# Autodesk Inventor assembly: P1704_E001
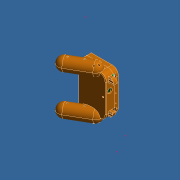
[picture p0: Inventor's stored thumbnail of the model, 180x180]
Saved by Autodesk Inventor 2019 (Build 230136000, 136)
## iProperties
Created: 2019-04-29
Part Number: P1704_E001
Material: Générique
Document SubType Name: Assembly
Designer: Joan.MAILLARD
Author: Joan.MAILLARD
## Documents named in this file (19)
- P:\projet_manette\manette\06_Dessins\2019\Manette universelle\P1704_E001.iam
- P:\projet_manette\manette\06_Dessins\2019\Manette universelle\P1704_001_basManette.ipt
- P:\projet_manette\manette\06_Dessins\2019\Manette universelle\P1704_006_gachette.ipt
- P:\projet_manette\manette\06_Dessins\2019\Manette universelle\P1704_007_guideRessort.ipt
- P:\projet_manette\manette\06_Dessins\2019\Manette universelle\P1704_002_mainDroiteInterieur.ipt
- P:\projet_manette\manette\06_Dessins\2019\Manette universelle\P1704_003_mainGaucheInterieur.ipt
- P:\projet_manette\manette\06_Dessins\2019\Manette universelle\P1704_009_slider.ipt
- P:\projet_manette\manette\06_Dessins\2019\Manette universelle\P1704_011_4buttonPCB.ipt
- P:\projet_manette\manette\06_Dessins\2019\Manette universelle\P1704_010_startSelectPCB.ipt
- P:\projet_manette\manette\06_Dessins\2019\Manette universelle\P1704_012_joystick.ipt
- P:\projet_manette\manette\06_Dessins\2019\Manette universelle\P1704_014_Display.ipt
- P:\projet_manette\manette\06_Dessins\2019\Manette universelle\P1704_015_rumble.ipt
- P:\projet_manette\manette\06_Dessins\2019\Manette universelle\P1704_008_pcb.ipt
- P:\projet_manette\manette\06_Dessins\2019\Manette universelle\P1704_018_hautManette.ipt
- P:\projet_manette\manette\06_Dessins\2019\Manette universelle\P1704_E003_button.iam
- P:\projet_manette\manette\06_Dessins\2019\Manette universelle\P1704_016_Button.ipt
- P:\projet_manette\manette\06_Dessins\2019\Manette universelle\P1704_019_button_triangle_cap.ipt
- P:\projet_manette\manette\06_Dessins\2019\Manette universelle\P1704_013_Switch.ipt
- P:\projet_manette\manette\06_Dessins\2019\Manette universelle\P1704_004_mainDroiteExterieur.ipt
## Components (37 placed, 18 different names)
1. P1704_001_basManette:1 — Placage:20, Placage:22, Placage:24, Placage:26, Placage:27, Placage:30, Placage:31, Placage:32, Placage:33, Placage:34, Placage:35, Placage:38, Placage:41, Placage:42, Placage:43, Placage:49, Affleurement:4, Affleurement:5, Placage:97, Affleurement:6, Placage:98, Placage:99, Placage:100, Placage:101, Placage:102, Placage:103, Placage:104, Placage:110, Placage:113, Placage:115, Placage:116, Placage:117, Placage:120
2. P1704_006_gachette:1 — Rotation:2, Glissière:4, Placage:26, Placage:27, Affleurement:1
3. P1704_006_gachette:2 — Rotation:1, Glissière:3, Affleurement:7, Placage:120
4. P1704_007_guideRessort:1 — Rotation:1
5. P1704_007_guideRessort:2 — Rotation:2
6. P1704_002_mainDroiteInterieur:1 — Placage:110, Placage:114, Placage:118
7. P1704_003_mainGaucheInterieur:1 — Placage:104, Placage:111, Placage:112
8. P1704_009_slider:1 — Glissière:3, Affleurement:7
9. P1704_009_slider:2 — Glissière:4, Affleurement:1
10. manette_2019_boutons.kicad_pcb_Contour:1 — Placage:22, Placage:52, Placage:53, Placage:54, Placage:56, Angle:1, Angle:2, Placage:57, Placage:58, Placage:59, Placage:60, Angle:3, Placage:61, Placage:62, Placage:63, Angle:4, Placage:64, Placage:65, Affleurement:6
11. manette_2019_boutons.kicad_pcb_Contour:2 — Placage:20, Placage:66, Placage:67, Placage:68, Placage:69, Placage:70, Angle:5, Angle:6, Angle:7, Angle:8, Placage:71, Placage:72, Placage:73, Placage:74, Placage:75, Placage:76, Placage:77, Angle:9, Angle:10, Angle:11, Angle:12, Placage:86, Placage:97
12. Manette_2019_PCB_Central.kicad_pcb_Contour:1 — Placage:24, Placage:87, Placage:88, Placage:89, Placage:90, Placage:91, Angle:13, Angle:14, Placage:92, Placage:93, Angle:15, Placage:98
13. P1704_012_joystick:1 — Placage:30, Placage:31, Placage:48
14. P1704_012_joystick:2 — Placage:32, Placage:33, Placage:47
15. P1704_014_Display:1 — Placage:38, Placage:50, Placage:96
16. P1704_015_rumble:1 — Placage:34, Placage:102
17. P1704_015_rumble:2 — Placage:35, Placage:103
18. manette_2019.kicad_pcb_Contour:1 — Placage:41, Placage:42, Placage:43, Placage:47, Placage:48
19. P1704_018_hautManette:1 — Placage:49, Affleurement:4, Affleurement:5, Placage:50, Placage:65, Placage:86, Placage:87, Placage:96
20. P1704_E003_button:1 [sub-assembly] — Placage:56, Angle:2, Placage:57, Placage:58
21. P1704_E003_button:2 [sub-assembly] — Placage:52, Placage:53, Placage:54, Angle:1
22. P1704_E003_button:3 [sub-assembly] — Placage:59, Placage:63, Angle:4, Placage:64
23. P1704_E003_button:4 [sub-assembly] — Placage:60, Angle:3, Placage:61, Placage:62
24. P1704_016_Button:1 — Placage:68, Angle:7, Placage:76, Placage:77, Placage:84, Placage:85
25. P1704_016_Button:2 — Placage:66, Angle:8, Placage:74, Placage:75, Placage:82, Placage:83
26. P1704_016_Button:3 — Placage:69, Angle:6, Placage:72, Placage:73, Placage:80, Placage:81
27. P1704_016_Button:4 — Placage:67, Placage:70, Angle:5, Placage:71, Placage:78, Placage:79
28. P1704_019_button_triangle_cap:1 — Placage:82, Placage:83, Angle:12
29. P1704_019_button_triangle_cap:2 — Placage:84, Placage:85, Angle:11
30. P1704_019_button_triangle_cap:3 — Placage:78, Placage:79, Angle:10
31. P1704_019_button_triangle_cap:4 — Placage:80, Placage:81, Angle:9
32. P1704_019_button_triangle_cap:5 — Placage:94, Placage:95, Angle:15
33. P1704_E003_button:5 [sub-assembly] — Placage:89, Placage:91, Angle:13, Placage:92
34. P1704_016_Button:5 — Placage:88, Placage:90, Angle:14, Placage:93, Placage:94, Placage:95
35. P1704_013_Switch:1 — Placage:99, Placage:100, Placage:101
36. P1704_004_mainDroiteExterieur:1 — Placage:111, Placage:112, Placage:113, Placage:116
37. P1704_004_mainDroiteExterieur:2 — Placage:114, Placage:115, Placage:117, Placage:118
## Relationships (105: Mate 81, Angle 15, Flush 5, RevoluteJoint 2, TranslationJoint 2)
- Rotation:1 [RevoluteJoint] (4.5 mm): P1704_006_gachette:2 ↔ P1704_007_guideRessort:1
- Rotation:2 [RevoluteJoint] (4.5 mm): P1704_006_gachette:1 ↔ P1704_007_guideRessort:2
- Glissière:3 [TranslationJoint]: P1704_006_gachette:2 ↔ P1704_009_slider:1
- Glissière:4 [TranslationJoint]: P1704_006_gachette:1 ↔ P1704_009_slider:2
- Placage:20 [Mate] (10 mm): P1704_001_basManette:1 ↔ manette_2019_boutons.kicad_pcb_Contour:2
- Placage:22 [Mate] (5 mm): P1704_001_basManette:1 ↔ manette_2019_boutons.kicad_pcb_Contour:1
- Placage:24 [Mate] (57.5375 mm): P1704_001_basManette:1 ↔ Manette_2019_PCB_Central.kicad_pcb_Contour:1
- Placage:26 [Mate]: P1704_001_basManette:1 ↔ P1704_006_gachette:1
- Placage:27 [Mate]: P1704_001_basManette:1 ↔ P1704_006_gachette:1
- Affleurement:1 [Flush]: P1704_006_gachette:1 ↔ P1704_009_slider:2
- Placage:30 [Mate] (35 mm): P1704_001_basManette:1 ↔ P1704_012_joystick:1
- Placage:31 [Mate] (40 mm): P1704_001_basManette:1 ↔ P1704_012_joystick:1
- Placage:32 [Mate] (35 mm): P1704_001_basManette:1 ↔ P1704_012_joystick:2
- Placage:33 [Mate] (35 mm): P1704_001_basManette:1 ↔ P1704_012_joystick:2
- Placage:34 [Mate]: P1704_001_basManette:1 ↔ P1704_015_rumble:1
- Placage:35 [Mate]: P1704_001_basManette:1 ↔ P1704_015_rumble:2
- Placage:38 [Mate] (53.375 mm): P1704_001_basManette:1 ↔ P1704_014_Display:1
- Placage:41 [Mate]: P1704_001_basManette:1 ↔ manette_2019.kicad_pcb_Contour:1
- Placage:42 [Mate]: P1704_001_basManette:1 ↔ manette_2019.kicad_pcb_Contour:1
- Placage:43 [Mate]: P1704_001_basManette:1 ↔ manette_2019.kicad_pcb_Contour:1
- Placage:47 [Mate] (7 mm): P1704_012_joystick:2 ↔ manette_2019.kicad_pcb_Contour:1
- Placage:48 [Mate] (7 mm): P1704_012_joystick:1 ↔ manette_2019.kicad_pcb_Contour:1
- Placage:49 [Mate]: P1704_001_basManette:1 ↔ P1704_018_hautManette:1
- Affleurement:4 [Flush]: P1704_001_basManette:1 ↔ P1704_018_hautManette:1
- Affleurement:5 [Flush]: P1704_001_basManette:1 ↔ P1704_018_hautManette:1
- Placage:50 [Mate]: P1704_014_Display:1 ↔ P1704_018_hautManette:1
- Placage:52 [Mate]: manette_2019_boutons.kicad_pcb_Contour:1 ↔ P1704_E003_button:2
- Placage:53 [Mate] (-37.465 mm): manette_2019_boutons.kicad_pcb_Contour:1 ↔ P1704_E003_button:2
- Placage:54 [Mate] (-19.05 mm): manette_2019_boutons.kicad_pcb_Contour:1 ↔ P1704_E003_button:2
- Placage:56 [Mate] (-24.765 mm): manette_2019_boutons.kicad_pcb_Contour:1 ↔ P1704_E003_button:1
- Angle:1 (0 deg): manette_2019_boutons.kicad_pcb_Contour:1 ↔ P1704_E003_button:2
- Angle:2 (0 deg): manette_2019_boutons.kicad_pcb_Contour:1 ↔ P1704_E003_button:1
- Placage:57 [Mate]: manette_2019_boutons.kicad_pcb_Contour:1 ↔ P1704_E003_button:1
- Placage:58 [Mate] (-30.48 mm): manette_2019_boutons.kicad_pcb_Contour:1 ↔ P1704_E003_button:1
- Placage:59 [Mate]: manette_2019_boutons.kicad_pcb_Contour:1 ↔ P1704_E003_button:3
- Placage:60 [Mate]: manette_2019_boutons.kicad_pcb_Contour:1 ↔ P1704_E003_button:4
- Angle:3 (0 deg): manette_2019_boutons.kicad_pcb_Contour:1 ↔ P1704_E003_button:4
- Placage:61 [Mate] (-24.765 mm): manette_2019_boutons.kicad_pcb_Contour:1 ↔ P1704_E003_button:4
- Placage:62 [Mate] (-7.62 mm): manette_2019_boutons.kicad_pcb_Contour:1 ↔ P1704_E003_button:4
- Placage:63 [Mate] (-12.065 mm): manette_2019_boutons.kicad_pcb_Contour:1 ↔ P1704_E003_button:3
- Angle:4 (0 deg): manette_2019_boutons.kicad_pcb_Contour:1 ↔ P1704_E003_button:3
- Placage:64 [Mate] (-19.05 mm): manette_2019_boutons.kicad_pcb_Contour:1 ↔ P1704_E003_button:3
- Placage:65 [Mate] (10 mm): manette_2019_boutons.kicad_pcb_Contour:1 ↔ P1704_018_hautManette:1
- Placage:66 [Mate]: manette_2019_boutons.kicad_pcb_Contour:2 ↔ P1704_016_Button:2
- Placage:67 [Mate]: manette_2019_boutons.kicad_pcb_Contour:2 ↔ P1704_016_Button:4
- Placage:68 [Mate]: manette_2019_boutons.kicad_pcb_Contour:2 ↔ P1704_016_Button:1
- Placage:69 [Mate]: manette_2019_boutons.kicad_pcb_Contour:2 ↔ P1704_016_Button:3
- Placage:70 [Mate] (-7.62 mm): manette_2019_boutons.kicad_pcb_Contour:2 ↔ P1704_016_Button:4
- Angle:5 (0 deg): manette_2019_boutons.kicad_pcb_Contour:2 ↔ P1704_016_Button:4
- Angle:6 (0 deg): manette_2019_boutons.kicad_pcb_Contour:2 ↔ P1704_016_Button:3
- Angle:7 (0 deg): manette_2019_boutons.kicad_pcb_Contour:2 ↔ P1704_016_Button:1
- Angle:8 (0 deg): manette_2019_boutons.kicad_pcb_Contour:2 ↔ P1704_016_Button:2
- Placage:71 [Mate] (-24.765 mm): manette_2019_boutons.kicad_pcb_Contour:2 ↔ P1704_016_Button:4
- Placage:72 [Mate] (-12.065 mm): manette_2019_boutons.kicad_pcb_Contour:2 ↔ P1704_016_Button:3
- Placage:73 [Mate] (-19.05 mm): manette_2019_boutons.kicad_pcb_Contour:2 ↔ P1704_016_Button:3
- Placage:74 [Mate] (-30.48 mm): manette_2019_boutons.kicad_pcb_Contour:2 ↔ P1704_016_Button:2
- Placage:75 [Mate] (-24.765 mm): manette_2019_boutons.kicad_pcb_Contour:2 ↔ P1704_016_Button:2
- Placage:76 [Mate] (-37.465 mm): manette_2019_boutons.kicad_pcb_Contour:2 ↔ P1704_016_Button:1
- Placage:77 [Mate] (-19.05 mm): manette_2019_boutons.kicad_pcb_Contour:2 ↔ P1704_016_Button:1
- Placage:78 [Mate]: P1704_016_Button:4 ↔ P1704_019_button_triangle_cap:3
- Placage:79 [Mate]: P1704_016_Button:4 ↔ P1704_019_button_triangle_cap:3
- Placage:80 [Mate]: P1704_016_Button:3 ↔ P1704_019_button_triangle_cap:4
- Placage:81 [Mate]: P1704_016_Button:3 ↔ P1704_019_button_triangle_cap:4
- Placage:82 [Mate]: P1704_016_Button:2 ↔ P1704_019_button_triangle_cap:1
- Placage:83 [Mate]: P1704_016_Button:2 ↔ P1704_019_button_triangle_cap:1
- Placage:84 [Mate]: P1704_016_Button:1 ↔ P1704_019_button_triangle_cap:2
- Placage:85 [Mate]: P1704_016_Button:1 ↔ P1704_019_button_triangle_cap:2
- Angle:9 (180 deg): manette_2019_boutons.kicad_pcb_Contour:2 ↔ P1704_019_button_triangle_cap:4
- Angle:10 (180 deg): manette_2019_boutons.kicad_pcb_Contour:2 ↔ P1704_019_button_triangle_cap:3
- Angle:11 (180 deg): manette_2019_boutons.kicad_pcb_Contour:2 ↔ P1704_019_button_triangle_cap:2
- Angle:12 (180 deg): manette_2019_boutons.kicad_pcb_Contour:2 ↔ P1704_019_button_triangle_cap:1
- Placage:86 [Mate] (10 mm): manette_2019_boutons.kicad_pcb_Contour:2 ↔ P1704_018_hautManette:1
- Placage:87 [Mate] (10 mm): Manette_2019_PCB_Central.kicad_pcb_Contour:1 ↔ P1704_018_hautManette:1
- Placage:88 [Mate]: Manette_2019_PCB_Central.kicad_pcb_Contour:1 ↔ P1704_016_Button:5
- Placage:89 [Mate]: Manette_2019_PCB_Central.kicad_pcb_Contour:1 ↔ P1704_E003_button:5
- Placage:90 [Mate] (-8.128 mm): Manette_2019_PCB_Central.kicad_pcb_Contour:1 ↔ P1704_016_Button:5
- Placage:91 [Mate] (-8.128 mm): Manette_2019_PCB_Central.kicad_pcb_Contour:1 ↔ P1704_E003_button:5
- Angle:13 (0 deg): Manette_2019_PCB_Central.kicad_pcb_Contour:1 ↔ P1704_E003_button:5
- Angle:14 (0 deg): Manette_2019_PCB_Central.kicad_pcb_Contour:1 ↔ P1704_016_Button:5
- Placage:92 [Mate] (-8.636 mm): Manette_2019_PCB_Central.kicad_pcb_Contour:1 ↔ P1704_E003_button:5
- Placage:93 [Mate] (-28.321 mm): Manette_2019_PCB_Central.kicad_pcb_Contour:1 ↔ P1704_016_Button:5
- Placage:94 [Mate]: P1704_019_button_triangle_cap:5 ↔ P1704_016_Button:5
- Placage:95 [Mate]: P1704_019_button_triangle_cap:5 ↔ P1704_016_Button:5
- Angle:15 (180 deg): Manette_2019_PCB_Central.kicad_pcb_Contour:1 ↔ P1704_019_button_triangle_cap:5
- Placage:96 [Mate] (0.5 mm): P1704_014_Display:1 ↔ P1704_018_hautManette:1
- Placage:97 [Mate] (58 mm): P1704_001_basManette:1 ↔ manette_2019_boutons.kicad_pcb_Contour:2
- Affleurement:6 [Flush] (45 mm): P1704_001_basManette:1 ↔ manette_2019_boutons.kicad_pcb_Contour:1
- Placage:98 [Mate] (55 mm): P1704_001_basManette:1 ↔ Manette_2019_PCB_Central.kicad_pcb_Contour:1
- Placage:99 [Mate]: P1704_001_basManette:1 ↔ P1704_013_Switch:1
- Placage:100 [Mate] (5 mm): P1704_001_basManette:1 ↔ P1704_013_Switch:1
- Placage:101 [Mate] (50 mm): P1704_001_basManette:1 ↔ P1704_013_Switch:1
- Placage:102 [Mate]: P1704_001_basManette:1 ↔ P1704_015_rumble:1
- Placage:103 [Mate]: P1704_001_basManette:1 ↔ P1704_015_rumble:2
- Placage:104 [Mate]: P1704_001_basManette:1 ↔ P1704_003_mainGaucheInterieur:1
- Placage:110 [Mate]: P1704_001_basManette:1 ↔ P1704_002_mainDroiteInterieur:1
- Placage:111 [Mate]: P1704_003_mainGaucheInterieur:1 ↔ P1704_004_mainDroiteExterieur:1
- Placage:112 [Mate]: P1704_003_mainGaucheInterieur:1 ↔ P1704_004_mainDroiteExterieur:1
- Placage:113 [Mate]: P1704_001_basManette:1 ↔ P1704_004_mainDroiteExterieur:1
- Placage:114 [Mate]: P1704_002_mainDroiteInterieur:1 ↔ P1704_004_mainDroiteExterieur:2
- Placage:115 [Mate]: P1704_001_basManette:1 ↔ P1704_004_mainDroiteExterieur:2
- Placage:116 [Mate]: P1704_001_basManette:1 ↔ P1704_004_mainDroiteExterieur:1
- Placage:117 [Mate]: P1704_001_basManette:1 ↔ P1704_004_mainDroiteExterieur:2
- Placage:118 [Mate]: P1704_002_mainDroiteInterieur:1 ↔ P1704_004_mainDroiteExterieur:2
- Affleurement:7 [Flush]: P1704_006_gachette:2 ↔ P1704_009_slider:1
- Placage:120 [Mate]: P1704_001_basManette:1 ↔ P1704_006_gachette:2
